# Autodesk Inventor assembly: poleStandHorizAssyB
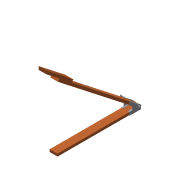
[picture p0: Inventor's stored thumbnail of the model, 180x180]
Saved by Autodesk Inventor 2016 SP2 (Build 200236200, 236)
## iProperties
Created: 2014-08-25
Part Number: poleStandHorizAssyB
Document SubType Name: Assembly
Designer: Dave
Author: Dave
## Documents named in this file (6)
- C:\Users\krosie\Google Drive\HERA\hera-cad\support\pole\poleStandHorizAssy.iam
- C:\Users\krosie\Google Drive\HERA\hera-cad\support\pole\poleStandHoriz2.ipt
- C:\Users\krosie\Google Drive\HERA\hera-cad\support\pole\poleStand37.ipt
- C:\Users\krosie\Google Drive\HERA\hera-cad\support\pole\poleStandHoriz3.ipt
- C:\Users\krosie\Google Drive\HERA\hera-cad\support\endcaps\HERA_end_cap_left.iam
- C:\Users\krosie\Google Drive\HERA\hera-cad\support\endcaps\HERA_end_cap_right.iam
## Components (5 placed, 5 different names)
1. HERA_end_cap_left:1 [sub-assembly] — Mate:9, Mate:10, Flush:3, Mate:11, Mate:12, Flush:4
2. poleStandHoriz2:1 — Mate:9, Mate:10, Flush:3
3. poleStand37:1 — Mate:11, Mate:12, Flush:4, Mate:13, Mate:14, Flush:5, Mate:15, Flush:6
4. poleStandHoriz3:1 — Mate:15, Flush:6
5. HERA_end_cap_right:1 [sub-assembly] — Mate:13, Mate:14, Flush:5
## Relationships (11: Mate 7, Flush 4)
- Mate:9: HERA_end_cap_left:1 ↔ poleStandHoriz2:1
- Mate:10: HERA_end_cap_left:1 ↔ poleStandHoriz2:1
- Flush:3 (37 mm): HERA_end_cap_left:1 ↔ poleStandHoriz2:1
- Mate:11: HERA_end_cap_left:1 ↔ poleStand37:1
- Mate:12: HERA_end_cap_left:1 ↔ poleStand37:1
- Flush:4: HERA_end_cap_left:1 ↔ poleStand37:1
- Mate:13: poleStand37:1 ↔ HERA_end_cap_right:1
- Mate:14: poleStand37:1 ↔ HERA_end_cap_right:1
- Flush:5: poleStand37:1 ↔ HERA_end_cap_right:1
- Mate:15: poleStand37:1 ↔ poleStandHoriz3:1
- Flush:6: poleStand37:1 ↔ poleStandHoriz3:1
